# Autodesk Inventor assembly: SUBReserviorPistonRod
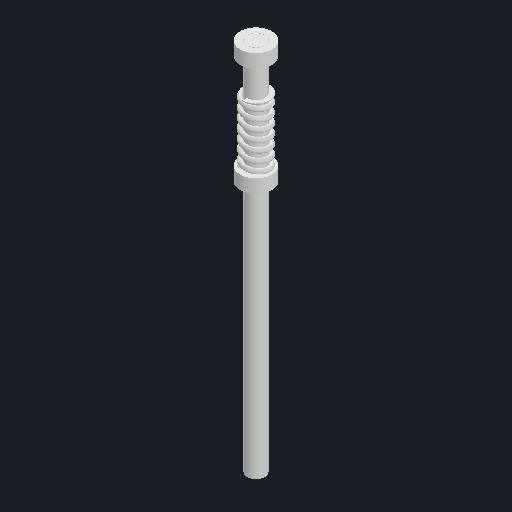
[picture p0: Inventor's stored thumbnail of the model, 512x512]
Saved by Autodesk Inventor 2024 (Build 280153000, 153)
## iProperties
Created: 2025-02-12
Part Number: SUBReserviorPistonRod
Document SubType Name: Assembly
Designer: Tommy Rohmann
Author: Tommy Rohmann
## Documents named in this file (4)
- C:\Users\Tommy Rohmann\OneDrive\Projects\Microgravity-Press-Washing-Machine\System Design and Documentation\Inventor Design Project\SUBReserviorPistonRod.iam
- C:\Users\Tommy Rohmann\OneDrive\Projects\Microgravity-Press-Washing-Machine\System Design and Documentation\Inventor Design Project\Compression Spring.ipt
- C:\Users\Tommy Rohmann\OneDrive\Projects\Microgravity-Press-Washing-Machine\System Design and Documentation\Inventor Design Project\ReserviorPistonRod.ipt
- C:\Users\Tommy Rohmann\OneDrive\Projects\Microgravity-Press-Washing-Machine\System Design and Documentation\Inventor Design Project\ShaftCollarReserviorPistonRod.ipt
## Components (4 placed, 3 different names)
1. Compression Spring:1 — Mate:1, Mate:4
2. ReserviorPistonRod:1 — Mate:1, Mate:2, Flush:1, Mate:3, Flush:2
3. ShaftCollarReserviorPistonRod:1 — Mate:2, Flush:1
4. ShaftCollarReserviorPistonRod:2 — Mate:3, Flush:2, Mate:4
## Relationships (6: Mate 4, Flush 2)
- Mate:1: Compression Spring:1 ↔ ReserviorPistonRod:1
- Mate:2: ReserviorPistonRod:1 ↔ ShaftCollarReserviorPistonRod:1
- Flush:1: ReserviorPistonRod:1 ↔ ShaftCollarReserviorPistonRod:1
- Mate:3: ReserviorPistonRod:1 ↔ ShaftCollarReserviorPistonRod:2
- Flush:2 (76.2 mm): ReserviorPistonRod:1 ↔ ShaftCollarReserviorPistonRod:2
- Mate:4: Compression Spring:1 ↔ ShaftCollarReserviorPistonRod:2
